# Autodesk Inventor assembly: CLQAM20
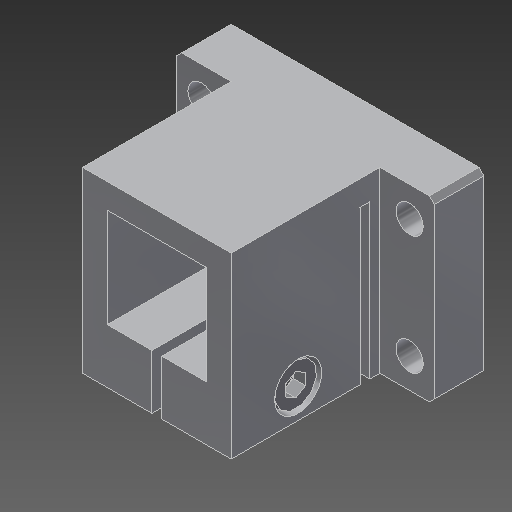
[picture p0: Inventor's stored thumbnail of the model, 512x512]
Saved by Autodesk Inventor 2021.1 (Build 251245010, 245A)
## iProperties
Created: 2010-03-11
Part Number: CLQAM20
Document SubType Name: Assembly
Title: スタンドブラケット
## Documents named in this file (3)
- Z:\inventorroom\sample\unit4\CLQAM20\CLQAM20.iam
- Z:\inventorroom\sample\unit4\CLQAM20\CLQAM20.ipt
- Z:\inventorroom\sample\unit4\CLQAM20\CBM5_18.ipt
## Components (2 placed, 2 different names)
1. CLQAM20:1 — 挿入:1
2. CBM5-18:1 — 挿入:1
## Relationships (1: Insert 1)
- 挿入:1 [Insert]: CLQAM20:1 ↔ CBM5-18:1
